# Autodesk Inventor assembly: EnsamblajeReal
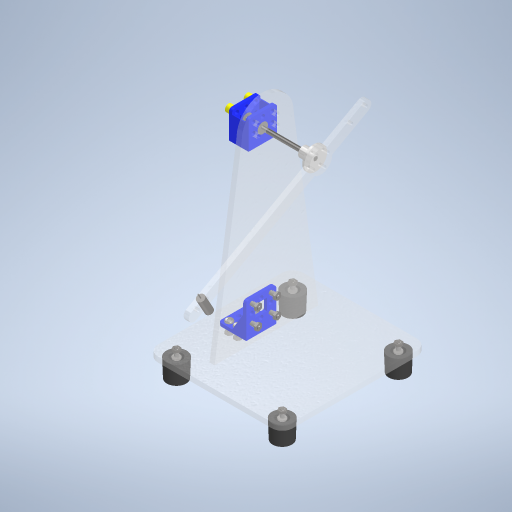
[picture p0: Inventor's stored thumbnail of the model, 512x512]
Saved by Autodesk Inventor 2023.1 (Build 271208000, 208)
## iProperties
Created: 2023-05-04
Part Number: EnsamblajeReal
Document SubType Name: Assembly
Designer: felip
Author: felip
## Documents named in this file (15)
- C:\Users\felip\OneDrive\UNAL FORE\SEMESTRE 9\TECNICAS DE CONTROL\PROYECTO\PROYECTO-TDC-INVENTOR\EnsamblajeReal.iam
- C:\Users\felip\OneDrive\UNAL FORE\SEMESTRE 9\TECNICAS DE CONTROL\PROYECTO\PROYECTO-TDC-INVENTOR\base.ipt
- C:\Users\felip\OneDrive\UNAL FORE\SEMESTRE 9\TECNICAS DE CONTROL\PROYECTO\PROYECTO-TDC-INVENTOR\Pata-Goma.ipt
- C:\Users\felip\OneDrive\Documents\Inventor\Content Center Files\R2023\en-US\BS 4183(7)\BS 4183 - M3,5 x 7(2) III.ipt
- C:\Users\felip\OneDrive\Documents\Inventor\Content Center Files\R2023\en-US\BS 4183(1)\BS 4183 - M3,5(1).ipt
- C:\Users\felip\OneDrive\UNAL FORE\SEMESTRE 9\TECNICAS DE CONTROL\PROYECTO\PROYECTO-TDC-INVENTOR\SoporteUnion.ipt
- C:\Users\felip\OneDrive\Documents\Inventor\Content Center Files\R2023\en-US\BS 4183(4)\BS 4183 - M3,5 x 11(1) III.ipt
- C:\Users\felip\OneDrive\UNAL FORE\SEMESTRE 9\TECNICAS DE CONTROL\PROYECTO\PROYECTO-TDC-INVENTOR\BaseParal.ipt
- C:\Users\felip\OneDrive\UNAL FORE\SEMESTRE 9\TECNICAS DE CONTROL\PROYECTO\PROYECTO-TDC-INVENTOR\SoporteEncoder.ipt
- C:\Users\felip\OneDrive\UNAL FORE\SEMESTRE 9\TECNICAS DE CONTROL\PROYECTO\PROYECTO-TDC-INVENTOR\rodamiento.ipt
- C:\Users\felip\OneDrive\UNAL FORE\SEMESTRE 9\TECNICAS DE CONTROL\PROYECTO\PROYECTO-TDC-INVENTOR\topito.ipt
- C:\Users\felip\OneDrive\UNAL FORE\SEMESTRE 9\TECNICAS DE CONTROL\PROYECTO\PROYECTO-TDC-INVENTOR\brida.ipt
- C:\Users\felip\OneDrive\UNAL FORE\SEMESTRE 9\TECNICAS DE CONTROL\PROYECTO\PROYECTO-TDC-INVENTOR\eje.ipt
- C:\Users\felip\OneDrive\UNAL FORE\SEMESTRE 9\TECNICAS DE CONTROL\PROYECTO\PROYECTO-TDC-INVENTOR\brazo.ipt
- C:\Users\felip\OneDrive\UNAL FORE\SEMESTRE 9\TECNICAS DE CONTROL\PROYECTO\PROYECTO-TDC-INVENTOR\motor.ipt
## Components (40 placed, 14 different names)
1. base:1 — Mate:1, Rotational:1, Mate:2, Mate:3, Mate:4, Rotational:2, Rotational:3, Mate:5, Rotational:4, Insert:1, Insert:2, Insert:3, Insert:4, Insert:5, Insert:10, Insert:11, Insert:12, Mate:6, Rotational:5, Rotational:6, Mate:8, Mate:10, Mate:12, Mate:14, Mate:15
2. Pata-Goma:1 — Mate:1, Rotational:1
3. Pata-Goma:2 — Mate:2, Mate:5, Rotational:4
4. Pata-Goma:3 — Mate:4, Rotational:3
5. Pata-Goma:4 — Mate:3, Rotational:2
6. BS 4183 Slotted Pan Head Machine Screw - Metric M3,5 x 7:1 — Insert:1
7. BS 4183 Slotted Pan Head Machine Screw - Metric M3,5 x 7:2 — Insert:2
8. BS 4183 Slotted Pan Head Machine Screw - Metric M3,5 x 7:3 — Insert:3
9. BS 4183 Slotted Pan Head Machine Screw - Metric M3,5 x 7:4 — Insert:4
10. BS 4183 - Metric M3,5:1 — Insert:5
11. BS 4183 - Metric M3,5:6 — Insert:10
12. BS 4183 - Metric M3,5:7 — Insert:11
13. BS 4183 - Metric M3,5:8 — Insert:12
14. SoporteUnion:1 — Mate:6, Rotational:5, Rotational:6, Insert:13, Insert:15, Insert:16, Insert:17, Mate:16, Rigid:1, Insert:18, Insert:20, Insert:22, Insert:23
15. BS 4183 Specification for machine screws and machine screw nuts. Metric series - Metric M3,5 x 11:1 — Insert:13, Mate:9
16. BS 4183 Specification for machine screws and machine screw nuts. Metric series - Metric M3,5 x 11:3 — Insert:15, Mate:13
17. BS 4183 Specification for machine screws and machine screw nuts. Metric series - Metric M3,5 x 11:4 — Insert:16, Mate:7
18. BS 4183 Specification for machine screws and machine screw nuts. Metric series - Metric M3,5 x 11:5 — Insert:17, Mate:11
19. BS 4183 - Metric M3,5:9 — Mate:7, Mate:8
20. BS 4183 - Metric M3,5:10 — Mate:9, Mate:10
21. BS 4183 - Metric M3,5:11 — Mate:11, Mate:12
22. BS 4183 - Metric M3,5:12 — Mate:13, Mate:14
23. BaseParal:1 — Mate:15, Mate:16, Rigid:1, Insert:24, Insert:30, Insert:31, Insert:32, Mate:17, Rigid:2
24. BS 4183 Specification for machine screws and machine screw nuts. Metric series - Metric M3,5 x 11:6 — Insert:18
25. BS 4183 Specification for machine screws and machine screw nuts. Metric series - Metric M3,5 x 11:8 — Insert:20
26. BS 4183 Specification for machine screws and machine screw nuts. Metric series - Metric M3,5 x 11:10 — Insert:22
27. BS 4183 Specification for machine screws and machine screw nuts. Metric series - Metric M3,5 x 11:11 — Insert:23
28. BS 4183 - Metric M3,5:13 — Insert:24
29. BS 4183 - Metric M3,5:19 — Insert:30
30. BS 4183 - Metric M3,5:20 — Insert:31
31. BS 4183 - Metric M3,5:21 — Insert:32
32. SoporteEncoder:1 — Mate:17, Insert:33, Insert:34, Insert:35, Insert:36
33. rodamiento:1 — Insert:33, Rigid:2
34. rodamiento:2 — Insert:34, Rotational:7
35. topito:1 — Insert:36
36. topito:2 — Insert:35
37. brida:1 — Insert:37, Mate:18, Rotational:8, Rotational:9
38. eje:1 — Insert:37, Rotational:7
39. brazo:1 — Mate:18, Rotational:8, Rotational:9, Tangent:1, Flush:1, Angle:1, Tangent:2
40. motor:1 — Tangent:1, Flush:1, Mate:19
## Relationships (59: Insert 25, Mate 19, RevoluteJoint 9, WeldJoint 2, Tangent 2, Flush 1, Angle 1)
- Mate:1: base:1 ↔ Pata-Goma:1
- Rotational:1 [RevoluteJoint]: base:1 ↔ Pata-Goma:1
- Mate:2: base:1 ↔ Pata-Goma:2
- Mate:3: base:1 ↔ Pata-Goma:4
- Mate:4: base:1 ↔ Pata-Goma:3
- Rotational:2 [RevoluteJoint]: base:1 ↔ Pata-Goma:4
- Rotational:3 [RevoluteJoint]: base:1 ↔ Pata-Goma:3
- Mate:5: base:1 ↔ Pata-Goma:2
- Rotational:4 [RevoluteJoint]: base:1 ↔ Pata-Goma:2
- Insert:1: base:1 ↔ BS 4183 Slotted Pan Head Machine Screw - Metric M3,5 x 7:1
- Insert:2: base:1 ↔ BS 4183 Slotted Pan Head Machine Screw - Metric M3,5 x 7:2
- Insert:3: base:1 ↔ BS 4183 Slotted Pan Head Machine Screw - Metric M3,5 x 7:3
- Insert:4: base:1 ↔ BS 4183 Slotted Pan Head Machine Screw - Metric M3,5 x 7:4
- Insert:5: base:1 ↔ BS 4183 - Metric M3,5:1
- Insert:10: base:1 ↔ BS 4183 - Metric M3,5:6
- Insert:11: base:1 ↔ BS 4183 - Metric M3,5:7
- Insert:12: base:1 ↔ BS 4183 - Metric M3,5:8
- Mate:6: base:1 ↔ SoporteUnion:1
- Rotational:5 [RevoluteJoint]: base:1 ↔ SoporteUnion:1
- Rotational:6 [RevoluteJoint]: base:1 ↔ SoporteUnion:1
- Insert:13: SoporteUnion:1 ↔ BS 4183 Specification for machine screws and machine screw nuts. Metric series - Metric M3,5 x 11:1
- Insert:15: SoporteUnion:1 ↔ BS 4183 Specification for machine screws and machine screw nuts. Metric series - Metric M3,5 x 11:3
- Insert:16: SoporteUnion:1 ↔ BS 4183 Specification for machine screws and machine screw nuts. Metric series - Metric M3,5 x 11:4
- Insert:17: SoporteUnion:1 ↔ BS 4183 Specification for machine screws and machine screw nuts. Metric series - Metric M3,5 x 11:5
- Mate:7: BS 4183 Specification for machine screws and machine screw nuts. Metric series - Metric M3,5 x 11:4 ↔ BS 4183 - Metric M3,5:9
- Mate:8: base:1 ↔ BS 4183 - Metric M3,5:9
- Mate:9: BS 4183 Specification for machine screws and machine screw nuts. Metric series - Metric M3,5 x 11:1 ↔ BS 4183 - Metric M3,5:10
- Mate:10: base:1 ↔ BS 4183 - Metric M3,5:10
- Mate:11: BS 4183 Specification for machine screws and machine screw nuts. Metric series - Metric M3,5 x 11:5 ↔ BS 4183 - Metric M3,5:11
- Mate:12: base:1 ↔ BS 4183 - Metric M3,5:11
- Mate:13: BS 4183 Specification for machine screws and machine screw nuts. Metric series - Metric M3,5 x 11:3 ↔ BS 4183 - Metric M3,5:12
- Mate:14: base:1 ↔ BS 4183 - Metric M3,5:12
- Mate:15: base:1 ↔ BaseParal:1
- Mate:16: SoporteUnion:1 ↔ BaseParal:1
- Rigid:1 [WeldJoint]: SoporteUnion:1 ↔ BaseParal:1
- Insert:18: SoporteUnion:1 ↔ BS 4183 Specification for machine screws and machine screw nuts. Metric series - Metric M3,5 x 11:6
- Insert:20: SoporteUnion:1 ↔ BS 4183 Specification for machine screws and machine screw nuts. Metric series - Metric M3,5 x 11:8
- Insert:22: SoporteUnion:1 ↔ BS 4183 Specification for machine screws and machine screw nuts. Metric series - Metric M3,5 x 11:10
- Insert:23: SoporteUnion:1 ↔ BS 4183 Specification for machine screws and machine screw nuts. Metric series - Metric M3,5 x 11:11
- Insert:24: BaseParal:1 ↔ BS 4183 - Metric M3,5:13
- Insert:30: BaseParal:1 ↔ BS 4183 - Metric M3,5:19
- Insert:31: BaseParal:1 ↔ BS 4183 - Metric M3,5:20
- Insert:32: BaseParal:1 ↔ BS 4183 - Metric M3,5:21
- Mate:17: BaseParal:1 ↔ SoporteEncoder:1
- Insert:33: SoporteEncoder:1 ↔ rodamiento:1
- Insert:34: SoporteEncoder:1 ↔ rodamiento:2
- Rigid:2 [WeldJoint]: BaseParal:1 ↔ rodamiento:1
- Insert:35: SoporteEncoder:1 ↔ topito:2
- Insert:36: SoporteEncoder:1 ↔ topito:1
- Insert:37: brida:1 ↔ eje:1
- Rotational:7 [RevoluteJoint]: rodamiento:2 ↔ eje:1
- Mate:18: brida:1 ↔ brazo:1
- Rotational:8 [RevoluteJoint]: brida:1 ↔ brazo:1
- Rotational:9 [RevoluteJoint]: brida:1 ↔ brazo:1
- Tangent:1: brazo:1 ↔ motor:1
- Flush:1 (-7 mm): brazo:1 ↔ motor:1
- Angle:1 (0 deg): brazo:1
- Tangent:2: brazo:1
- Mate:19 (-5.5 mm): motor:1
